# Autodesk Inventor assembly: 189199 ESH-HA-4-QS---(0)
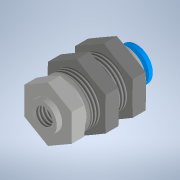
[picture p0: Inventor's stored thumbnail of the model, 180x180]
Saved by Autodesk Inventor 2021 (Build 250183000, 183)
## iProperties
Category: PARTsolutions
Company: FESTO
Created: 2026-04-19
Part Number: 189199 ESH-HA-4-QS---(0)
Catalog Web Link: www.3dfindit.com
Description: ESH-suction cup holder
Vendor: FESTO
Document SubType Name: Assembly
Designer: psAdmin
Manufacturer: FESTO
Mass: 30 g
Surface Area: 31.8741 cm^2
Volume: 4.16384 cm^3
Density: 7.20489 g/cm^3
Title: 189199 ESH-HA-4-QS
Author: Cadenas PARTsolutions
Comments: suction cup holder
PSOL_IDENT_0: {ATYP=ASSISTANT},{DATA=script=$CADENAS_DATA/23d-libs/festo/webfesto.vbb&M_FAMILY=ESH&M_GROUP=01&M_PA
PSOL_IDENT_1: RTNO=189199&IDCODE1=ESH-HA-4-QS&IDCODE2=&customer_number_cns=&MATES=1&LOD=HI&LOCKERP=0&SINGLEPART=1}
NB: 189199 ESH-HA-4-QS---(0)
NN: ESH
NT: suction cup holder
NBSYN: $TNR. $TYP.---($HUB.)
LINA: 189199 ESH-HA-4-QS
CATALOG: Festo
TNR: 189199
TYP: ESH-HA-4-QS
HUB: 0
CNSMASSEXACT: 0.03
GTIN: 4052568041663
REACH: Yes
REACHSVHC: Yes
REACHHAZSUBS: 7439-92-1
REACHVALDATE: 05.03.2025
SUPPLIER: FESTO
ARTICLENO: 189199 ESH-HA-4-QS---(0)
BOMINFO: 189199 ESH-HA-4-QS
CREATOR: CADENAS GmbH
## Documents named in this file (3)
- e:\temp\worker_COMMON_184\temp\tmp_592_20_1Wx8h\format_0\189199 ESH-HA-4-QS---(0).iam
- e:\temp\worker_COMMON_184\temp\tmp_592_20_1Wx8h\format_0\189199 ESH-HA-4-QS.ipt
- e:\temp\worker_COMMON_184\temp\tmp_592_20_1Wx8h\format_0\130519 ESHM-M14x1.ipt
## Components (3 placed, 2 different names)
1. 189199 ESH-HA-4-QS:1 — MUTTER1_Z@1 <-> ANBAU_Z@2, MUTTER1_YZ@1 <-> ANBAU_YZ@2, MUTTER2_Z@1 <-> ANBAU_Z@3, MUTTER2_YZ@1 <-> ANBAU_YZ@3
2. 130519 ESHM-M14x1:1 — MUTTER1_Z@1 <-> ANBAU_Z@2, MUTTER1_YZ@1 <-> ANBAU_YZ@2
3. 130519 ESHM-M14x1:2 — MUTTER2_Z@1 <-> ANBAU_Z@3, MUTTER2_YZ@1 <-> ANBAU_YZ@3
## Relationships (4: Mate 2, Angle 2)
- MUTTER1_Z@1 <-> ANBAU_Z@2 [Mate]: 189199 ESH-HA-4-QS:1 ↔ 130519 ESHM-M14x1:1
- MUTTER1_YZ@1 <-> ANBAU_YZ@2 [Angle] (0 deg): 189199 ESH-HA-4-QS:1 ↔ 130519 ESHM-M14x1:1
- MUTTER2_Z@1 <-> ANBAU_Z@3 [Mate]: 189199 ESH-HA-4-QS:1 ↔ 130519 ESHM-M14x1:2
- MUTTER2_YZ@1 <-> ANBAU_YZ@3 [Angle] (0 deg): 189199 ESH-HA-4-QS:1 ↔ 130519 ESHM-M14x1:2
